# Autodesk Inventor assembly: KapalPembersihLaut.0025
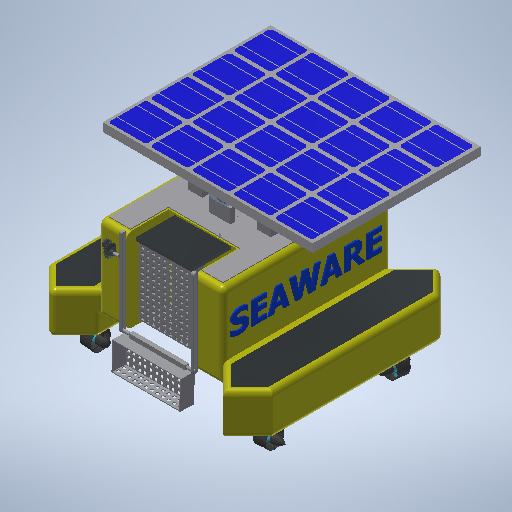
[picture p0: Inventor's stored thumbnail of the model, 512x512]
Saved by Autodesk Inventor 2025.2 (Build 292293000, 293)
## iProperties
Created: 2025-05-22
Part Number: KapalPembersihLaut.0025
Document SubType Name: Assembly
Designer: hando
ASRestoreLoc: D:\Data_Lokal\Kuliah\Tri Wahyu (22518241023)\Lomba Essay\Himpunan Administrasi Publik UNY\Design Kapal\KapalPembersihLaut.iam
Author: hando
## Documents named in this file (25)
- D:\Data_Lokal\Kuliah\Tri Wahyu (22518241023)\Lomba Essay\Himpunan Administrasi Publik UNY\Design Kapal\Autosave\KapalPembersihLaut.0025.iam
- D:\Data_Lokal\Kuliah\Tri Wahyu (22518241023)\Lomba Essay\Himpunan Administrasi Publik UNY\Design Kapal\diamond-dynamics-thruster-1-2kg-1.snapshot.3\Thrusters v13\Thrusters v13\Thrusters v13.iam
- D:\Data_Lokal\Kuliah\Tri Wahyu (22518241023)\Lomba Essay\Himpunan Administrasi Publik UNY\Design Kapal\Base.ipt
- D:\Data_Lokal\Kuliah\Tri Wahyu (22518241023)\Lomba Essay\Himpunan Administrasi Publik UNY\Design Kapal\pg-36-dc-motor-1.snapshot.2\PG36.ipt
- D:\Data_Lokal\Kuliah\Tri Wahyu (22518241023)\Lomba Essay\Himpunan Administrasi Publik UNY\Design Kapal\bracket-pg36-1.snapshot.2\brecket encoder\brecket encoder\brecket encoder.ipt
- D:\Data_Lokal\Kuliah\Tri Wahyu (22518241023)\Lomba Essay\Himpunan Administrasi Publik UNY\Design Kapal\WadahSampah.ipt
- D:\Data_Lokal\Kuliah\Tri Wahyu (22518241023)\Lomba Essay\Himpunan Administrasi Publik UNY\Design Kapal\Solar panel.ipt
- D:\Data_Lokal\Kuliah\Tri Wahyu (22518241023)\Lomba Essay\Himpunan Administrasi Publik UNY\Design Kapal\Wadah+Solar.ipt
- D:\Data_Lokal\Kuliah\Tri Wahyu (22518241023)\Lomba Essay\Himpunan Administrasi Publik UNY\Design Kapal\Logitech c270 Assembly.iam
- D:\Data_Lokal\Kuliah\Tri Wahyu (22518241023)\Lomba Essay\Himpunan Administrasi Publik UNY\Design Kapal\Pengangkut.ipt
- D:\Data_Lokal\Kuliah\Tri Wahyu (22518241023)\Lomba Essay\Himpunan Administrasi Publik UNY\Design Kapal\KapalPembersihLaut\Design Accelerator\Bevel Gears1.iam
- D:\Data_Lokal\Kuliah\Tri Wahyu (22518241023)\Lomba Essay\Himpunan Administrasi Publik UNY\Design Kapal\KapalPembersihLaut\Design Accelerator\Bevel Gears2.iam
- D:\Data_Lokal\Kuliah\Tri Wahyu (22518241023)\Lomba Essay\Himpunan Administrasi Publik UNY\Design Kapal\Pemilah.ipt
- D:\Data_Lokal\Kuliah\Tri Wahyu (22518241023)\Lomba Essay\Himpunan Administrasi Publik UNY\Design Kapal\raspberry-pi-5-2.snapshot.8\RASPBERRY_PI_5\RASPBERRY_PI_5\RASPBERRY_PI_5.iam
- D:\Data_Lokal\Kuliah\Tri Wahyu (22518241023)\Lomba Essay\Himpunan Administrasi Publik UNY\Design Kapal\driverbtn v1.iam
- D:\Data_Lokal\Kuliah\Tri Wahyu (22518241023)\Lomba Essay\Himpunan Administrasi Publik UNY\Design Kapal\Pejal.ipt
- D:\Data_Lokal\Kuliah\Tri Wahyu (22518241023)\Lomba Essay\Himpunan Administrasi Publik UNY\Design Kapal\Jalur Pejal.ipt
- D:\Data_Lokal\Kuliah\Tri Wahyu (22518241023)\Lomba Essay\Himpunan Administrasi Publik UNY\Design Kapal\bevel-gear-217.snapshot.1\Bevel Gear 1\Bevel Gear 1\Bevel Gear 1.ipt
- D:\Data_Lokal\Kuliah\Tri Wahyu (22518241023)\Lomba Essay\Himpunan Administrasi Publik UNY\Design Kapal\Penyambung Jalur Pejal.ipt
- D:\Data_Lokal\Kuliah\Tri Wahyu (22518241023)\Lomba Essay\Himpunan Administrasi Publik UNY\Design Kapal\mg90-micro-servo-1.snapshot.5\MG90servo_assembly\MG90servo_assembly\MG90servo_assembly.iam
- D:\Data_Lokal\Kuliah\Tri Wahyu (22518241023)\Lomba Essay\Himpunan Administrasi Publik UNY\Design Kapal\BATERIA.ipt
- D:\Data_Lokal\Kuliah\Tri Wahyu (22518241023)\Lomba Essay\Himpunan Administrasi Publik UNY\Design Kapal\neo-6m-gps-module-1.snapshot.2\neo6mGps\neo6mGps\neo6mGps.ipt
- D:\Data_Lokal\Kuliah\Tri Wahyu (22518241023)\Lomba Essay\Himpunan Administrasi Publik UNY\Design Kapal\Penutup Pelampung.ipt
- D:\Data_Lokal\Kuliah\Tri Wahyu (22518241023)\Lomba Essay\Himpunan Administrasi Publik UNY\Design Kapal\ph-sensor-1.snapshot.1\pH_Sensor\pH_Sensor\pH_Sensor.iam
- D:\Data_Lokal\Kuliah\Tri Wahyu (22518241023)\Lomba Essay\Himpunan Administrasi Publik UNY\Design Kapal\dfrobot-gravity-dissolved-oxygen-sensor-v1-0-1.snapshot.1\Gravity Dissolved Oxygen Sensor v1.0\Gravity Diss.ipt
## Components (34 placed, 23 different names)
1. Thrusters v13:2 [sub-assembly] — Flush:7, Flush:8
2. Base:1 — Flush:1, Flush:2, Flush:3, Flush:4, Flush:5, Flush:6, Flush:7, Flush:8, Mate:8, Mate:9, Mate:10, Mate:11, Mate:15, Mate:16, Mate:19, Mate:20, Mate:23, Flush:14, Flush:15, Mate:25, Flush:17, Flush:18, Flush:19, Mate:31, Mate:32, Mate:33, Mate:34, Cylindrical:1, Cylindrical:2
3. Thrusters v13:3 [sub-assembly] — Flush:1, Flush:2
4. Thrusters v13:4 [sub-assembly] — Flush:3, Flush:4
5. Thrusters v13:5 [sub-assembly] — Flush:5, Flush:6
6. PG36:1 — Mate:3, Mate:4, Rotational:2
7. brecket encoder:1 — Mate:3, Mate:4, Mate:9, Mate:10, Mate:11
8. WadahSampah:1 — Mate:8, Flush:19
9. Solar panel:1 — Flush:11, Flush:12, Mate:17
10. Wadah+Solar:1 — Mate:15, Mate:16, Flush:11, Flush:12, Mate:17, Mate:21, Mate:22, Mate:28, Flush:20, Mate:29, Mate:30, Mate:35, Mate:36, Mate:37, Mate:38
11. Logitech c270 Assembly:1 [sub-assembly] — Mate:30
12. Pengangkut:1 — Rotational:1
13. Bevel Gears:1 [sub-assembly]
14. Bevel Gears:2 [sub-assembly]
15. Pemilah:1 — Mate:19, Mate:20, Rotational:3
16. RASPBERRY_PI_5:1 [sub-assembly] — Mate:21
17. driverbtn v1:1 [sub-assembly] — Mate:22
18. Pejal:1 — Slider:1, Rotational:1
19. Jalur Pejal:1 — Mate:23, Flush:14, Flush:15, Slider:1
20. Jalur Pejal:2 — Mate:25, Flush:17, Flush:18
21. Bevel Gear 1:1 — Rotational:2
22. Bevel Gear 1:2 — Mate:26, Mate:27
23. Penyambung Jalur Pejal:1 — Mate:26, Mate:27
24. MG90servo_assembly:1 [sub-assembly] — Rotational:3
25. BATERIA:1 — Mate:28, Flush:20
26. neo6mGps:1 — Mate:29
27. Penutup Pelampung:1 — Mate:31, Mate:32
28. Penutup Pelampung:2 — Mate:33, Mate:34
29. pH_Sensor:1 [sub-assembly] — Cylindrical:1
30. Gravity Diss:1 — Cylindrical:2
31. driverbtn v1:2 [sub-assembly] — Mate:37
32. driverbtn v1:3 [sub-assembly] — Mate:36
33. driverbtn v1:4 [sub-assembly] — Mate:38
34. driverbtn v1:5 [sub-assembly] — Mate:35
## Relationships (50: Mate 28, Flush 16, RevoluteJoint 3, CylindricalJoint 2, TranslationJoint 1)
- Flush:1 (5 mm): Base:1 ↔ Thrusters v13:3
- Flush:2 (3.5 mm): Base:1 ↔ Thrusters v13:3
- Flush:3 (3.5 mm): Base:1 ↔ Thrusters v13:4
- Flush:4 (5 mm): Base:1 ↔ Thrusters v13:4
- Flush:5 (5 mm): Base:1 ↔ Thrusters v13:5
- Flush:6 (3.5 mm): Base:1 ↔ Thrusters v13:5
- Flush:7 (5 mm): Thrusters v13:2 ↔ Base:1
- Flush:8 (3.5 mm): Thrusters v13:2 ↔ Base:1
- Mate:3: PG36:1 ↔ brecket encoder:1
- Mate:4: PG36:1 ↔ brecket encoder:1
- Mate:8: Base:1 ↔ WadahSampah:1
- Mate:9: Base:1 ↔ brecket encoder:1
- Mate:10: Base:1 ↔ brecket encoder:1
- Mate:11 (20 mm): Base:1 ↔ brecket encoder:1
- Mate:15: Base:1 ↔ Wadah+Solar:1
- Mate:16: Base:1 ↔ Wadah+Solar:1
- Flush:11 (-170 mm): Solar panel:1 ↔ Wadah+Solar:1
- Flush:12 (-190 mm): Solar panel:1 ↔ Wadah+Solar:1
- Mate:17: Solar panel:1 ↔ Wadah+Solar:1
- Mate:19: Base:1 ↔ Pemilah:1
- Mate:20: Base:1 ↔ Pemilah:1
- Mate:21: Wadah+Solar:1 ↔ RASPBERRY_PI_5:1
- Mate:22: Wadah+Solar:1 ↔ driverbtn v1:1
- Mate:23: Base:1 ↔ Jalur Pejal:1
- Flush:14: Base:1 ↔ Jalur Pejal:1
- Flush:15 (-10 mm): Base:1 ↔ Jalur Pejal:1
- Mate:25: Base:1 ↔ Jalur Pejal:2
- Flush:17 (-10 mm): Base:1 ↔ Jalur Pejal:2
- Flush:18: Base:1 ↔ Jalur Pejal:2
- Slider:1 [TranslationJoint] (125 mm): Pejal:1 ↔ Jalur Pejal:1
- Rotational:1 [RevoluteJoint] (-30 mm): Pengangkut:1 ↔ Pejal:1
- Rotational:2 [RevoluteJoint] (-10 mm): PG36:1 ↔ Bevel Gear 1:1
- Flush:19 (10 mm): Base:1 ↔ WadahSampah:1
- Mate:26: Bevel Gear 1:2 ↔ Penyambung Jalur Pejal:1
- Mate:27: Bevel Gear 1:2 ↔ Penyambung Jalur Pejal:1
- Rotational:3 [RevoluteJoint]: Pemilah:1 ↔ MG90servo_assembly:1
- Mate:28: Wadah+Solar:1 ↔ BATERIA:1
- Flush:20 (130 mm): Wadah+Solar:1 ↔ BATERIA:1
- Mate:29: Wadah+Solar:1 ↔ neo6mGps:1
- Mate:30 (10 mm): Wadah+Solar:1 ↔ Logitech c270 Assembly:1
- Mate:31: Base:1 ↔ Penutup Pelampung:1
- Mate:32: Base:1 ↔ Penutup Pelampung:1
- Mate:33: Base:1 ↔ Penutup Pelampung:2
- Mate:34: Base:1 ↔ Penutup Pelampung:2
- Cylindrical:1: Base:1 ↔ pH_Sensor:1
- Cylindrical:2: Base:1 ↔ Gravity Diss:1
- Mate:35: Wadah+Solar:1 ↔ driverbtn v1:5
- Mate:36: Wadah+Solar:1 ↔ driverbtn v1:3
- Mate:37: Wadah+Solar:1 ↔ driverbtn v1:2
- Mate:38: Wadah+Solar:1 ↔ driverbtn v1:4
